# Autodesk Inventor assembly: Assembly
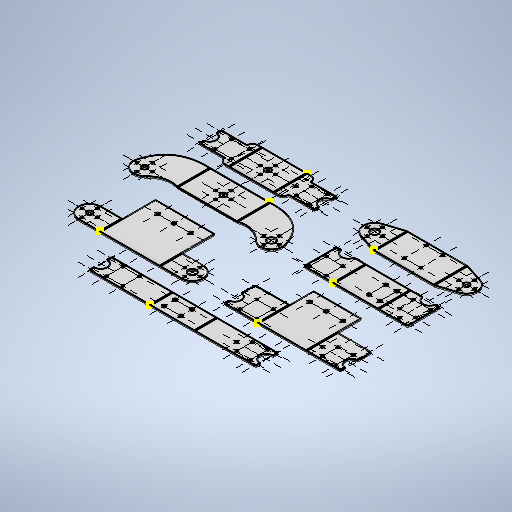
[picture p0: Inventor's stored thumbnail of the model, 512x512]
Saved by Autodesk Inventor 2025.2 (Build 292293000, 293)
## iProperties
Created: 2025-08-12
Part Number: Assembly
Document SubType Name: Assembly
Designer: LG
Author: LG
## Documents named in this file (8)
- C:\Users\LG\Desktop\RHp_Humanoid_ver1\CAM\Arm\Right Arm\1.5T\Assembly\Assembly.iam
- C:\Users\LG\Desktop\RHp_Humanoid_ver1\CAM\Arm\Right Arm\1.5T\Part\axis_18_top_frame.ipt
- C:\Users\LG\Desktop\RHp_Humanoid_ver1\CAM\Arm\Right Arm\1.5T\Part\axis_19_bottom_frame.ipt
- C:\Users\LG\Desktop\RHp_Humanoid_ver1\CAM\Arm\Right Arm\1.5T\Part\axis_20_bottom_frame.ipt
- C:\Users\LG\Desktop\RHp_Humanoid_ver1\CAM\Arm\Right Arm\1.5T\Part\axis_21_top_frame.ipt
- C:\Users\LG\Desktop\RHp_Humanoid_ver1\CAM\Arm\Right Arm\1.5T\Part\axis_21_bottom_frame.ipt
- C:\Users\LG\Desktop\RHp_Humanoid_ver1\CAM\Arm\Right Arm\1.5T\Part\axis_22_bottom_frame.ipt
- C:\Users\LG\Desktop\RHp_Humanoid_ver1\CAM\Arm\Right Arm\1.5T\Part\axis_22_top_frame.ipt
## Components (7 placed, 7 different names)
1. axis_18_top_frame:1 — Mate:1, Flush:1, Mate:2, Mate:3, Mate:4, Flush:2, Mate:5, Flush:3, Flush:4, Mate:6, Mate:7, Flush:5, Mate:8, Flush:6, Flush:7, Mate:9, Mate:10, Flush:8, Mate:11, Mate:12, Flush:9
2. axis_19_bottom_frame:1 — Mate:5, Flush:3, Flush:4
3. axis_20_bottom_frame:1 — Mate:3, Mate:4, Flush:2
4. axis_21_top_frame:1 — Mate:11, Mate:12, Flush:9
5. axis_21_bottom_frame:1 — Mate:6, Mate:7, Flush:5
6. axis_22_bottom_frame:1 — Mate:8, Flush:6, Flush:7
7. axis_22_top_frame:1 — Mate:9, Mate:10, Flush:8
## Relationships (21: Mate 12, Flush 9)
- Mate:1: axis_18_top_frame:1
- Flush:1: axis_18_top_frame:1
- Mate:2: axis_18_top_frame:1
- Mate:3 (10 mm): axis_18_top_frame:1 ↔ axis_20_bottom_frame:1
- Mate:4 (6 mm): axis_18_top_frame:1 ↔ axis_20_bottom_frame:1
- Flush:2: axis_18_top_frame:1 ↔ axis_20_bottom_frame:1
- Mate:5 (45 mm): axis_18_top_frame:1 ↔ axis_19_bottom_frame:1
- Flush:3: axis_18_top_frame:1 ↔ axis_19_bottom_frame:1
- Flush:4: axis_18_top_frame:1 ↔ axis_19_bottom_frame:1
- Mate:6 (40 mm): axis_18_top_frame:1 ↔ axis_21_bottom_frame:1
- Mate:7 (15 mm): axis_18_top_frame:1 ↔ axis_21_bottom_frame:1
- Flush:5: axis_18_top_frame:1 ↔ axis_21_bottom_frame:1
- Mate:8 (60 mm): axis_18_top_frame:1 ↔ axis_22_bottom_frame:1
- Flush:6 (-25 mm): axis_18_top_frame:1 ↔ axis_22_bottom_frame:1
- Flush:7: axis_18_top_frame:1 ↔ axis_22_bottom_frame:1
- Mate:9 (33 mm): axis_18_top_frame:1 ↔ axis_22_top_frame:1
- Mate:10 (60 mm): axis_18_top_frame:1 ↔ axis_22_top_frame:1
- Flush:8: axis_18_top_frame:1 ↔ axis_22_top_frame:1
- Mate:11 (125 mm): axis_18_top_frame:1 ↔ axis_21_top_frame:1
- Mate:12 (-55 mm): axis_18_top_frame:1 ↔ axis_21_top_frame:1
- Flush:9: axis_18_top_frame:1 ↔ axis_21_top_frame:1
